# Autodesk Inventor assembly: S8x2
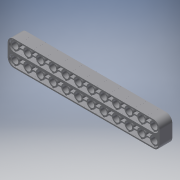
[picture p0: Inventor's stored thumbnail of the model, 180x180]
Saved by Autodesk Inventor 2019 (Build 230136000, 136)
## iProperties
Created: 2019-01-31
Part Number: S8x2
Document SubType Name: Assembly
Designer: Varga Daniel
Author: Varga Daniel
## Documents named in this file (3)
- C:\!_Dani\!_cloud\OneDrive\!_munka\Revolution\RevvyDemoKit\Structural parts\Straight Beams\S12x2.iam
- C:\!_Dani\!_cloud\OneDrive\!_munka\Revolution\RevvyDemoKit\Structural parts\Straight Beams\straight_beam_end_part_double.ipt
- C:\!_Dani\!_cloud\OneDrive\!_munka\Revolution\RevvyDemoKit\Structural parts\Straight Beams\straight_beam_inner_part_double.ipt
## Components (12 placed, 2 different names)
1. straight_beam_end_part_double:1 — Flush:8, Flush:9, Mate:2
2. straight_beam_end_part_double:2 — Mate:12, Flush:23, Flush:24
3. straight_beam_inner_part_double:1 — Flush:3, Flush:4, Flush:12, Flush:13, Mate:5, Mate:6
4. straight_beam_inner_part_double:2 — Flush:4, Flush:5, Flush:13, Flush:14, Mate:6, Mate:7
5. straight_beam_inner_part_double:3 — Flush:5, Flush:14, Mate:7, Flush:21, Flush:22, Mate:11
6. straight_beam_inner_part_double:4 — Flush:2, Flush:3, Flush:11, Flush:12, Mate:4, Mate:5
7. straight_beam_inner_part_double:5 — Flush:1, Flush:2, Flush:10, Flush:11, Mate:3, Mate:4
8. straight_beam_inner_part_double:6 — Flush:1, Flush:8, Flush:9, Mate:2, Flush:10, Mate:3
9. straight_beam_inner_part_double:7
10. straight_beam_inner_part_double:8
11. straight_beam_inner_part_double:9 — Mate:12, Flush:23, Flush:24
12. straight_beam_inner_part_double:10 — Flush:21, Flush:22, Mate:11
## Relationships (33: Flush 22, Mate 11)
- Flush:1: straight_beam_inner_part_double:5 ↔ straight_beam_inner_part_double:6
- Flush:2: straight_beam_inner_part_double:4 ↔ straight_beam_inner_part_double:5
- Flush:3: straight_beam_inner_part_double:1 ↔ straight_beam_inner_part_double:4
- Flush:4: straight_beam_inner_part_double:1 ↔ straight_beam_inner_part_double:2
- Flush:5: straight_beam_inner_part_double:2 ↔ straight_beam_inner_part_double:3
- Flush:8: straight_beam_end_part_double:1 ↔ straight_beam_inner_part_double:6
- Flush:9: straight_beam_end_part_double:1 ↔ straight_beam_inner_part_double:6
- Mate:2: straight_beam_end_part_double:1 ↔ straight_beam_inner_part_double:6
- Flush:10: straight_beam_inner_part_double:5 ↔ straight_beam_inner_part_double:6
- Flush:11: straight_beam_inner_part_double:4 ↔ straight_beam_inner_part_double:5
- Flush:12: straight_beam_inner_part_double:1 ↔ straight_beam_inner_part_double:4
- Flush:13: straight_beam_inner_part_double:1 ↔ straight_beam_inner_part_double:2
- Flush:14: straight_beam_inner_part_double:2 ↔ straight_beam_inner_part_double:3
- Mate:3: straight_beam_inner_part_double:5 ↔ straight_beam_inner_part_double:6
- Mate:4: straight_beam_inner_part_double:4 ↔ straight_beam_inner_part_double:5
- Mate:5: straight_beam_inner_part_double:1 ↔ straight_beam_inner_part_double:4
- Mate:6: straight_beam_inner_part_double:1 ↔ straight_beam_inner_part_double:2
- Mate:7: straight_beam_inner_part_double:2 ↔ straight_beam_inner_part_double:3
- [Flush]: straight_beam_inner_part_double:7 ↔ straight_beam_inner_part_double:10
- [Flush]: straight_beam_inner_part_double:7 ↔ straight_beam_inner_part_double:8
- [Flush]: straight_beam_inner_part_double:8 ↔ straight_beam_inner_part_double:9
- [Flush]: straight_beam_inner_part_double:7 ↔ straight_beam_inner_part_double:10
- [Flush]: straight_beam_inner_part_double:7 ↔ straight_beam_inner_part_double:8
- [Flush]: straight_beam_inner_part_double:8 ↔ straight_beam_inner_part_double:9
- [Mate]: straight_beam_inner_part_double:7 ↔ straight_beam_inner_part_double:10
- [Mate]: straight_beam_inner_part_double:7 ↔ straight_beam_inner_part_double:8
- [Mate]: straight_beam_inner_part_double:8 ↔ straight_beam_inner_part_double:9
- Flush:21: straight_beam_inner_part_double:3 ↔ straight_beam_inner_part_double:10
- Flush:22: straight_beam_inner_part_double:3 ↔ straight_beam_inner_part_double:10
- Mate:11: straight_beam_inner_part_double:3 ↔ straight_beam_inner_part_double:10
- Mate:12: straight_beam_end_part_double:2 ↔ straight_beam_inner_part_double:9
- Flush:23: straight_beam_end_part_double:2 ↔ straight_beam_inner_part_double:9
- Flush:24: straight_beam_end_part_double:2 ↔ straight_beam_inner_part_double:9
## Named parameters: d21_d13 = 0 mm, d22_d14 = 0 mm, d23_d15 = 0 mm, d24_d18 = 0 mm, d25_d19 = 0 mm, d26_d20 = 0 mm, d27_d2 = 0 mm, d28_d3 = 0 mm, d29_d4 = 0 mm
